# Autodesk Inventor assembly: SRM with Smoke Grain
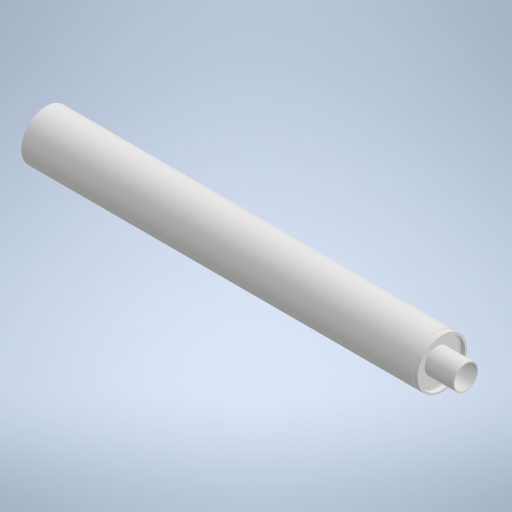
[picture p0: Inventor's stored thumbnail of the model, 512x512]
Saved by Autodesk Inventor 2024 (Build 280153000, 153)
## iProperties
Created: 2024-01-11
Part Number: SRM with Smoke Grain
Document SubType Name: Assembly
Designer: auror
Author: auror
## Documents named in this file (8)
- C:\Users\auror\Documents\TU Delft\DARE\Scrambler-II\SRM with Smoke Grain.iam
- C:\Users\auror\Documents\TU Delft\DARE\Solids\TRP-SRM2020\Grain.ipt
- C:\Users\auror\Documents\TU Delft\DARE\Solids\TRP-SRM2020\Spacer_ring.ipt
- C:\Users\auror\Documents\TU Delft\DARE\Scrambler-II\Smoke grain.ipt
- C:\Users\auror\Documents\TU Delft\DARE\Solids\TRP-SRM2020\SRM 2020 Casing EE5.ipt
- SRM 2020 Casing EE5.ipt
- C:\Users\auror\Documents\TU Delft\DARE\Solids\TRP-SRM2020\Nozzle.ipt
- C:\Users\auror\Documents\TU Delft\DARE\Solids\TRP-SRM2020\Endcap.ipt
## Components (14 placed, 6 different names)
1. Grain:1 — Mate:1, Mate:2, Mate:4, Mate:5, Mate:12, Mate:21
2. Grain:2 — Mate:3, Mate:4, Mate:6, Mate:7, Mate:8, Mate:10
3. Grain:3 — Mate:11, Mate:12, Mate:13, Mate:14, Mate:18
4. Grain:4 — Mate:9, Mate:10, Mate:15, Mate:16, Mate:20
5. Spacer_ring:1 — Mate:13, Mate:14, Mate:17
6. Spacer_ring:2 — Mate:1, Mate:2, Mate:3
7. Spacer_ring:3 — Mate:7, Mate:8, Mate:9
8. Spacer_ring:4 — Mate:5, Mate:6, Mate:11
9. Spacer_ring:5 — Mate:15, Mate:16
10. Smoke grain:1 — Mate:17, Mate:18, Mate:19, Mate:25
11. Spacer_ring:6 — Mate:19, Mate:20, Mate:24
12. SRM 2020 Casing EE5:1 — Mate:21, Mate:22, Mate:26, Mate:27
13. Nozzle:1 — Mate:22, Mate:27
14. Endcap:1 — Mate:24, Mate:25, Mate:26
## Relationships (26: Mate 26)
- Mate:1: Grain:1 ↔ Spacer_ring:2
- Mate:2: Grain:1 ↔ Spacer_ring:2
- Mate:3: Grain:2 ↔ Spacer_ring:2
- Mate:4: Grain:1 ↔ Grain:2
- Mate:5: Grain:1 ↔ Spacer_ring:4
- Mate:6: Grain:2 ↔ Spacer_ring:4
- Mate:7: Grain:2 ↔ Spacer_ring:3
- Mate:8: Grain:2 ↔ Spacer_ring:3
- Mate:9: Grain:4 ↔ Spacer_ring:3
- Mate:10: Grain:2 ↔ Grain:4
- Mate:11: Grain:3 ↔ Spacer_ring:4
- Mate:12: Grain:1 ↔ Grain:3
- Mate:13: Grain:3 ↔ Spacer_ring:1
- Mate:14: Grain:3 ↔ Spacer_ring:1
- Mate:15: Grain:4 ↔ Spacer_ring:5
- Mate:16: Grain:4 ↔ Spacer_ring:5
- Mate:17: Spacer_ring:1 ↔ Smoke grain:1
- Mate:18: Grain:3 ↔ Smoke grain:1
- Mate:19: Smoke grain:1 ↔ Spacer_ring:6
- Mate:20: Grain:4 ↔ Spacer_ring:6
- Mate:21: Grain:1 ↔ SRM 2020 Casing EE5:1
- Mate:22: SRM 2020 Casing EE5:1 ↔ Nozzle:1
- Mate:24: Spacer_ring:6 ↔ Endcap:1
- Mate:25: Smoke grain:1 ↔ Endcap:1
- Mate:26: SRM 2020 Casing EE5:1 ↔ Endcap:1
- Mate:27: SRM 2020 Casing EE5:1 ↔ Nozzle:1
